# Autodesk Inventor assembly: Gripper Attempt 04
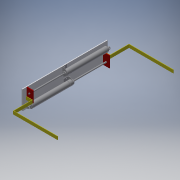
[picture p0: Inventor's stored thumbnail of the model, 180x180]
Saved by Autodesk Inventor 2016 (Build 200138000, 138)
## iProperties
Created: 2015-06-19
Part Number: Gripper Attempt 04
Document SubType Name: Assembly
Designer: steele
Author: steele
## Documents named in this file (8)
- C:\snobotics\CAD\robSteele\Gripper\Gripper Attempt 04.iam
- C:\snobotics\CAD\robSteele\ipart Components\Plate for Gripper\Plate for Gripper 6 x 27 x 1_4.ipt
- C:\snobotics\CAD\robSteele\ipart Components\Plate for Gripper.ipt
- C:\snobotics\CAD\partResources\McMaster-Carr\Air Cylinder\Pivot Mount Cylinders\Foot Bracket for 1_25 and 1_50 Bore\6498K340.ipt
- C:\snobotics\CAD\robSteele\ipart Components\Gripper Arm.ipt
- C:\snobotics\CAD\robSteele\Gripper\Gripper Piston.ipt
- C:\snobotics\CAD\partResources\McMaster-Carr\Air Cylinder\Pivot Mount Cylinders\Double Acting\Force 155 Bore 1_50\Stroke 10\6498K681.ipt
- C:\snobotics\CAD\robSteele\ipart Components\Gripper Arm\Gripper Arm 1 x 6 x 16 x 1_8.ipt
## Components (9 placed, 5 different names)
1. Plate for Gripper 6 x 27 x 1_4:1 — Mate:1, Flush:1, Flush:2, Mate:2, Flush:3, Flush:4, Flush:5
2. 6498K340:1 — Mate:2, Flush:3, Flush:4, Mate:7
3. 6498K340:2 — Mate:1, Flush:1, Flush:2, Mate:8
4. Gripper Arm 1 x 6 x 16 x 1_8:1 — Mate:6, Flush:8, Flush:9
5. Gripper Arm 1 x 6 x 16 x 1_8:2 — Mate:5, Flush:6, Flush:7
6. Gripper Piston:1 — Mate:5, Flush:6, Flush:7, Insert:1
7. Gripper Piston:2 — Flush:5, Mate:6, Flush:8, Flush:9, Insert:2
8. 6498K681:1 — Mate:7, Insert:1
9. 6498K681:2 — Mate:8, Insert:2
## Relationships (17: Flush 9, Mate 6, Insert 2)
- Mate:1: Plate for Gripper 6 x 27 x 1_4:1 ↔ 6498K340:2
- Flush:1: Plate for Gripper 6 x 27 x 1_4:1 ↔ 6498K340:2
- Flush:2 (330.2 mm): Plate for Gripper 6 x 27 x 1_4:1 ↔ 6498K340:2
- Mate:2: Plate for Gripper 6 x 27 x 1_4:1 ↔ 6498K340:1
- Flush:3: Plate for Gripper 6 x 27 x 1_4:1 ↔ 6498K340:1
- Flush:4 (330.2 mm): Plate for Gripper 6 x 27 x 1_4:1 ↔ 6498K340:1
- Flush:5: Plate for Gripper 6 x 27 x 1_4:1 ↔ Gripper Piston:2
- Mate:5: Gripper Arm 1 x 6 x 16 x 1_8:2 ↔ Gripper Piston:1
- Flush:6: Gripper Arm 1 x 6 x 16 x 1_8:2 ↔ Gripper Piston:1
- Flush:7: Gripper Arm 1 x 6 x 16 x 1_8:2 ↔ Gripper Piston:1
- Mate:6: Gripper Arm 1 x 6 x 16 x 1_8:1 ↔ Gripper Piston:2
- Flush:8: Gripper Arm 1 x 6 x 16 x 1_8:1 ↔ Gripper Piston:2
- Flush:9: Gripper Arm 1 x 6 x 16 x 1_8:1 ↔ Gripper Piston:2
- Mate:7: 6498K340:1 ↔ 6498K681:1
- Mate:8: 6498K340:2 ↔ 6498K681:2
- Insert:1 (-12.7 mm): Gripper Piston:1 ↔ 6498K681:1
- Insert:2 (-12.7 mm): Gripper Piston:2 ↔ 6498K681:2
## Named parameters: offsetToFrontOfAirCylinder = 330.2 mm
